# Autodesk Inventor assembly: CaseAssembly
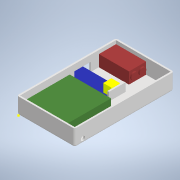
[picture p0: Inventor's stored thumbnail of the model, 180x180]
Saved by Autodesk Inventor 2021 (Build 250183000, 183)
## iProperties
Created: 2021-01-18
Part Number: CaseAssembly
Document SubType Name: Assembly
Designer: Jayan
Author: Jayan
## Documents named in this file (5)
- C:\Data\Jayanth\SchoolWork\FISD_FriscoHighSchool\10th_Grade_FHS\Science Fair\CaseAssembly.iam
- C:\Data\Jayanth\SchoolWork\FISD_FriscoHighSchool\10th_Grade_FHS\Science Fair\OuterCase.ipt
- C:\Data\Jayanth\SchoolWork\FISD_FriscoHighSchool\10th_Grade_FHS\Science Fair\ArduinoBoard.ipt
- C:\Data\Jayanth\SchoolWork\FISD_FriscoHighSchool\10th_Grade_FHS\Science Fair\PowerSource.ipt
- C:\Data\Jayanth\SchoolWork\FISD_FriscoHighSchool\10th_Grade_FHS\Science Fair\WaterSensor.ipt
## Components (4 placed, 4 different names)
1. OuterCase:1 — Mate:1, Mate:2, Mate:3, Mate:4, Mate:5, Mate:6, Mate:7, Flush:1
2. ArduinoBoard:2 — Mate:1, Mate:2, Mate:3
3. PowerSource:1 — Mate:4, Mate:5, Mate:6
4. WaterSensor:1 — Mate:7, Flush:1
## Relationships (8: Mate 7, Flush 1)
- Mate:1: OuterCase:1 ↔ ArduinoBoard:2
- Mate:2: OuterCase:1 ↔ ArduinoBoard:2
- Mate:3: OuterCase:1 ↔ ArduinoBoard:2
- Mate:4: OuterCase:1 ↔ PowerSource:1
- Mate:5: OuterCase:1 ↔ PowerSource:1
- Mate:6: OuterCase:1 ↔ PowerSource:1
- Mate:7: OuterCase:1 ↔ WaterSensor:1
- Flush:1: OuterCase:1 ↔ WaterSensor:1
